# Autodesk Inventor assembly: SchleppstangeKopf
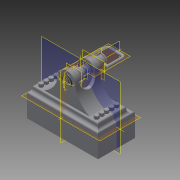
[picture p0: Inventor's stored thumbnail of the model, 180x180]
Saved by Autodesk Inventor 2015 (Build 190159000, 159)
## iProperties
Created: 2018-11-30
Part Number: SchleppstangeKopf
Document SubType Name: Assembly
Designer: Boris
Author: Boris
## Documents named in this file (5)
- D:\Wisag Hiserv\HiSERV Smart Drive\WorkOrder\3D - Teile\SchleppstangeKopf.iam
- D:\Wisag Hiserv\HiSERV Smart Drive\WorkOrder\3D - Teile\SchleppstangeBefestigung.ipt
- D:\Wisag Hiserv\HiSERV Smart Drive\WorkOrder\3D - Teile\SchleppstangeBefestigungOben.ipt
- D:\Wisag Hiserv\HiSERV Smart Drive\WorkOrder\3D - Teile\SchleppstangeBefestigungUnten.ipt
- D:\Wisag Hiserv\HiSERV Smart Drive\WorkOrder\3D - Teile\SchleppstangeHauptTeil.ipt
## Components (4 placed, 4 different names)
1. SchleppstangeBefestigung:1 — Einfügen:2
2. SchleppstangeBefestigungOben:1 — Einfügen:3
3. SchleppstangeBefestigungUnten:1 — Einfügen:1, Einfügen:2
4. SchleppstangeHauptTeil:1 — Einfügen:1, Einfügen:3
## Relationships (3: Insert 3)
- Einfügen:1 [Insert] (-2 mm): SchleppstangeBefestigungUnten:1 ↔ SchleppstangeHauptTeil:1
- Einfügen:2 [Insert] (-3 mm): SchleppstangeBefestigung:1 ↔ SchleppstangeBefestigungUnten:1
- Einfügen:3 [Insert] (-2 mm): SchleppstangeBefestigungOben:1 ↔ SchleppstangeHauptTeil:1
